# Autodesk Inventor assembly: 自由輪部分
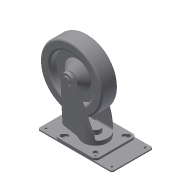
[picture p0: Inventor's stored thumbnail of the model, 180x180]
Saved by Autodesk Inventor 2020.3 (Build 243373000, 373)
## iProperties
Part Number: 自由輪部分
Material: 一般
Document SubType Name: Assembly
Designer: highs
Author: highs
## Documents named in this file (3)
- C:\Users\toshi\Desktop\中の島ex\自由輪部分.iam
- C:\Users\toshi\Desktop\中の島ex\自由輪.iam
- C:\Users\toshi\Desktop\中の島ex\自由輪マウント.ipt
## Components (2 placed, 2 different names)
1. 自由輪:1 [sub-assembly] — メイト:1, メイト:2, メイト:3
2. 自由輪マウント:1 — メイト:1, メイト:2, メイト:3
## Relationships (3: Mate 3)
- メイト:1 [Mate]: 自由輪:1 ↔ 自由輪マウント:1
- メイト:2 [Mate]: 自由輪:1 ↔ 自由輪マウント:1
- メイト:3 [Mate]: 自由輪:1 ↔ 自由輪マウント:1
